# Autodesk Inventor assembly: Shooter Mount6000
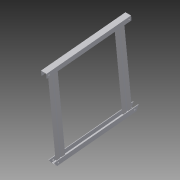
[picture p0: Inventor's stored thumbnail of the model, 180x180]
Saved by Autodesk Inventor 2013 (Build 170138000, 138)
## iProperties
Created: 2013-01-09
Part Number: Shooter Mount6000
Document SubType Name: Assembly
Designer: Naphat
Author: Naphat
## Documents named in this file (4)
- C:\Users\carneeki\Desktop\Kiwi Robot\Rack\Rack.iam
- C:\Users\carneeki\Desktop\Kiwi Robot\Rack\Rack - Back.ipt
- C:\Users\carneeki\Desktop\Kiwi Robot\Rack\Rack - Front.ipt
- C:\Users\carneeki\Desktop\Kiwi Robot\Rack\Rack - Cross Members.ipt
## Components (4 placed, 3 different names)
1. Rack - Back:1 — Mate:1, Mate:2, Mate:5, Mate:6, Insert:3
2. Rack - Front:1 — Mate:3, Mate:4, Mate:7, Insert:1, Insert:2
3. Rack - Cross Members:1 — Mate:5, Mate:6, Mate:7, Insert:2, Insert:3
4. Rack - Cross Members:2 — Mate:1, Mate:2, Mate:3, Mate:4, Insert:1
## Relationships (10: Mate 7, Insert 3)
- Mate:1: Rack - Back:1 ↔ Rack - Cross Members:2
- Mate:2: Rack - Back:1 ↔ Rack - Cross Members:2
- Mate:3: Rack - Front:1 ↔ Rack - Cross Members:2
- Mate:4: Rack - Front:1 ↔ Rack - Cross Members:2
- Mate:5: Rack - Back:1 ↔ Rack - Cross Members:1
- Mate:6: Rack - Back:1 ↔ Rack - Cross Members:1
- Mate:7: Rack - Front:1 ↔ Rack - Cross Members:1
- Insert:1: Rack - Front:1 ↔ Rack - Cross Members:2
- Insert:2: Rack - Front:1 ↔ Rack - Cross Members:1
- Insert:3: Rack - Back:1 ↔ Rack - Cross Members:1
